# Autodesk Inventor assembly: Arbor Press Assembly
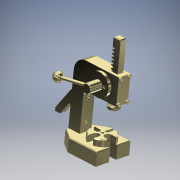
[picture p0: Inventor's stored thumbnail of the model, 180x180]
Saved by Autodesk Inventor 2018 (Build 220112000, 112)
## iProperties
Created: 2018-01-09
Part Number: Arbor Press Assembly
Document SubType Name: Assembly
Designer: 232963
Author: 232963
## Documents named in this file (16)
- P:\IED\Arbor Press\Arbor Press Assembly.iam
- P:\IED\Arbor Press\Base.ipt
- P:\IED\Arbor Press\Column.ipt
- P:\IED\Arbor Press\8-32 UNC Bolt.ipt
- P:\IED\Arbor Press\3-8-16 UNC Bolt.ipt
- P:\IED\Arbor Press\Gear.ipt
- P:\IED\Arbor Press\Gear Rack.ipt
- P:\IED\Arbor Press\Handle.ipt
- P:\IED\Arbor Press\Handle Cover Plate.ipt
- P:\IED\Arbor Press\Gear Plate.ipt
- P:\IED\Arbor Press\Cover Plate.ipt
- P:\IED\Arbor Press\Rack Pad.ipt
- P:\IED\Arbor Press\Table.ipt
- P:\IED\Arbor Press\Table Pin.ipt
- P:\IED\Arbor Press\Punch Holder.ipt
- P:\IED\Arbor Press\8-32 UNC Flathead Bolt.ipt
## Components (24 placed, 15 different names)
1. Base:1 — Rigid:1, Mate:1, Mate:19, Mate:20, Insert:1
2. Column:1 — Rigid:1, Mate:1, Mate:3, Mate:4, Mate:5, Mate:6, Mate:10, Mate:14, Mate:15, Mate:16, Insert:2, Insert:3, Insert:4, Insert:8, Insert:9, Insert:10, Mate:21, Insert:17
3. 8-32 UNC Bolt:1 — Insert:13
4. 3-8-16 UNC Bolt:1 — Insert:4
5. Gear:1 — Mate:3, Mate:4, Rotation/Translation:1, Mate:7, Mate:8, Flush:2
6. Gear Rack:1 — Mate:5, Mate:6, Rotation/Translation:1, Mate:17, Mate:18
7. Handle:1 — Mate:7, Mate:8, Flush:2, Mate:9
8. Handle Cover Plate:1 — Mate:9, Mate:10, Insert:10, Insert:11, Insert:12
9. Gear Plate:1 — Mate:21, Insert:17
10. Cover Plate:1 — Mate:14, Mate:15, Mate:16, Insert:13, Insert:14, Insert:15, Insert:16
11. Rack Pad:1 — Mate:17, Mate:18
12. Table:1 — Insert:1
13. Table Pin:1 — Mate:19, Mate:20
14. Punch Holder:1 — Insert:2, Insert:3
15. 8-32 UNC Bolt:2
16. 8-32 UNC Bolt:3
17. 8-32 UNC Bolt:4 — Insert:12
18. 8-32 UNC Bolt:5
19. 8-32 UNC Bolt:6 — Insert:11
20. 8-32 UNC Bolt:7 — Insert:15
21. 8-32 UNC Bolt:8 — Insert:14
22. 8-32 UNC Bolt:9 — Insert:16
23. 8-32 UNC Flathead Bolt:1 — Insert:8
24. 8-32 UNC Flathead Bolt:2 — Insert:9
## Relationships (34: Mate 17, Insert 14, WeldJoint 1, RelateRotateTranslate 1, Flush 1)
- Rigid:1 [WeldJoint]: Base:1 ↔ Column:1
- Mate:1: Base:1 ↔ Column:1
- Mate:3: Column:1 ↔ Gear:1
- Mate:4: Column:1 ↔ Gear:1
- Mate:5: Column:1 ↔ Gear Rack:1
- Mate:6: Column:1 ↔ Gear Rack:1
- Rotation/Translation:1 [RelateRotateTranslate] (79.248 mm): Gear:1 ↔ Gear Rack:1
- Mate:7: Gear:1 ↔ Handle:1
- Mate:8: Gear:1 ↔ Handle:1
- Flush:2: Gear:1 ↔ Handle:1
- Mate:9: Handle:1 ↔ Handle Cover Plate:1
- Mate:10: Column:1 ↔ Handle Cover Plate:1
- Mate:14: Column:1 ↔ Cover Plate:1
- Mate:15: Column:1 ↔ Cover Plate:1
- Mate:16: Column:1 ↔ Cover Plate:1
- Mate:17: Gear Rack:1 ↔ Rack Pad:1
- Mate:18: Gear Rack:1 ↔ Rack Pad:1
- Mate:19: Base:1 ↔ Table Pin:1
- Mate:20: Base:1 ↔ Table Pin:1
- Insert:1: Base:1 ↔ Table:1
- Insert:2: Column:1 ↔ Punch Holder:1
- Insert:3: Column:1 ↔ Punch Holder:1
- Insert:4: Column:1 ↔ 3-8-16 UNC Bolt:1
- Insert:8: Column:1 ↔ 8-32 UNC Flathead Bolt:1
- Insert:9: Column:1 ↔ 8-32 UNC Flathead Bolt:2
- Insert:10: Column:1 ↔ Handle Cover Plate:1
- Insert:11: Handle Cover Plate:1 ↔ 8-32 UNC Bolt:6
- Insert:12: Handle Cover Plate:1 ↔ 8-32 UNC Bolt:4
- Insert:13: 8-32 UNC Bolt:1 ↔ Cover Plate:1
- Insert:14: Cover Plate:1 ↔ 8-32 UNC Bolt:8
- Insert:15: Cover Plate:1 ↔ 8-32 UNC Bolt:7
- Insert:16: Cover Plate:1 ↔ 8-32 UNC Bolt:9
- Mate:21: Column:1 ↔ Gear Plate:1
- Insert:17: Column:1 ↔ Gear Plate:1
